# Autodesk Inventor assembly: Assembly1
(part 4 of 8)
- [Mate]: disk holder:94 ↔ Coil:188
- [Angle] (270 deg): disk holder:94 ↔ Coil:188
- [Mate]: disk holder:94 ↔ Coil:188
- [RevoluteJoint]: disk holder:95 ↔ coin:95
- [Angle] (-25 deg): disk holder:95 ↔ coin:95
- [Mate]: disk holder:95 ↔ Coil:189
- [Mate]: disk holder:95 ↔ Coil:189
- [Angle] (270 deg): disk holder:95 ↔ Coil:189
- [Mate]: disk holder:95 ↔ Coil:190
- [Angle] (270 deg): disk holder:95 ↔ Coil:190
- [Mate]: disk holder:95 ↔ Coil:190
- [RevoluteJoint]: disk holder:96 ↔ coin:96
- [Angle] (-25 deg): disk holder:96 ↔ coin:96
- [Mate]: disk holder:96 ↔ Coil:191
- [Mate]: disk holder:96 ↔ Coil:191
- [Angle] (270 deg): disk holder:96 ↔ Coil:191
- [Mate]: disk holder:96 ↔ Coil:192
- [Angle] (270 deg): disk holder:96 ↔ Coil:192
- [Mate]: disk holder:96 ↔ Coil:192
- [RevoluteJoint]: disk holder:97 ↔ coin:97
- [Angle] (-25 deg): disk holder:97 ↔ coin:97
- [Mate]: disk holder:97 ↔ Coil:193
- [Mate]: disk holder:97 ↔ Coil:193
- [Angle] (270 deg): disk holder:97 ↔ Coil:193
- [Mate]: disk holder:97 ↔ Coil:194
- [Angle] (270 deg): disk holder:97 ↔ Coil:194
- [Mate]: disk holder:97 ↔ Coil:194
- [RevoluteJoint]: disk holder:98 ↔ coin:98
- [Angle] (-25 deg): disk holder:98 ↔ coin:98
- [Mate]: disk holder:98 ↔ Coil:195
- [Mate]: disk holder:98 ↔ Coil:195
- [Angle] (270 deg): disk holder:98 ↔ Coil:195
- [Mate]: disk holder:98 ↔ Coil:196
- [Angle] (270 deg): disk holder:98 ↔ Coil:196
- [Mate]: disk holder:98 ↔ Coil:196
- [RevoluteJoint]: disk holder:99 ↔ coin:99
- [Angle] (-25 deg): disk holder:99 ↔ coin:99
- [Mate]: disk holder:99 ↔ Coil:197
- [Mate]: disk holder:99 ↔ Coil:197
- [Angle] (270 deg): disk holder:99 ↔ Coil:197
- [Mate]: disk holder:99 ↔ Coil:198
- [Angle] (270 deg): disk holder:99 ↔ Coil:198
- [Mate]: disk holder:99 ↔ Coil:198
- [RevoluteJoint]: disk holder:100 ↔ coin:100
- [Angle] (-25 deg): disk holder:100 ↔ coin:100
- [Mate]: disk holder:100 ↔ Coil:199
- [Mate]: disk holder:100 ↔ Coil:199
- [Angle] (270 deg): disk holder:100 ↔ Coil:199
- [Mate]: disk holder:100 ↔ Coil:200
- [Angle] (270 deg): disk holder:100 ↔ Coil:200
- [Mate]: disk holder:100 ↔ Coil:200
- [RevoluteJoint]: disk holder:101 ↔ coin:101
- [Angle] (-25 deg): disk holder:101 ↔ coin:101
- [Mate]: disk holder:101 ↔ Coil:201
- [Mate]: disk holder:101 ↔ Coil:201
- [Angle] (270 deg): disk holder:101 ↔ Coil:201
- [Mate]: disk holder:101 ↔ Coil:202
- [Angle] (270 deg): disk holder:101 ↔ Coil:202
- [Mate]: disk holder:101 ↔ Coil:202
- [RevoluteJoint]: disk holder:102 ↔ coin:102
- [Angle] (-25 deg): disk holder:102 ↔ coin:102
- [Mate]: disk holder:102 ↔ Coil:203
- [Mate]: disk holder:102 ↔ Coil:203
- [Angle] (270 deg): disk holder:102 ↔ Coil:203
- [Mate]: disk holder:102 ↔ Coil:204
- [Angle] (270 deg): disk holder:102 ↔ Coil:204
- [Mate]: disk holder:102 ↔ Coil:204
- Flush:135: FRAME:1 ↔ disk holder:94
- Mate:559: FRAME:1 ↔ disk holder:94
- Flush:136: disk holder:92 ↔ disk holder:94
- Flush:137: disk holder:92 ↔ disk holder:94
- Flush:138: disk holder:92 ↔ disk holder:93
- Flush:139: disk holder:92 ↔ disk holder:93
- Flush:140: disk holder:93 ↔ disk holder:95
- Flush:141: disk holder:93 ↔ disk holder:95
- Flush:142: disk holder:95 ↔ disk holder:96
- Flush:143: disk holder:95 ↔ disk holder:97
- Flush:144: disk holder:97 ↔ disk holder:98
- Flush:145: disk holder:98 ↔ disk holder:99
- Flush:146: disk holder:99 ↔ disk holder:100
- Flush:147: disk holder:95 ↔ disk holder:101
- Flush:148: disk holder:101 ↔ disk holder:102
- Flush:149: disk holder:93 ↔ disk holder:96
- Flush:150: disk holder:95 ↔ disk holder:97
- Flush:151: disk holder:95 ↔ disk holder:98
- Flush:152: disk holder:99 ↔ disk holder:100
- Flush:153: disk holder:100 ↔ disk holder:101
- Flush:154: disk holder:101 ↔ disk holder:102
- Flush:155: disk holder:98 ↔ disk holder:99
- Mate:560: FRAME:1 ↔ disk holder:94
- Mate:561: FRAME:1 ↔ disk holder:92
- Mate:562: FRAME:1 ↔ disk holder:93
- Mate:563: FRAME:1 ↔ disk holder:96
- Mate:564: FRAME:1 ↔ disk holder:97
- Mate:565: FRAME:1 ↔ disk holder:95
- Mate:566: FRAME:1 ↔ disk holder:98
- Mate:567: FRAME:1 ↔ disk holder:99
- Mate:568: FRAME:1 ↔ disk holder:100
- Mate:569: FRAME:1 ↔ disk holder:101
- Mate:570: FRAME:1 ↔ disk holder:102
- [RevoluteJoint]: disk holder:103 ↔ coin:103
- [Angle] (-25 deg): disk holder:103 ↔ coin:103
- [Mate]: disk holder:103 ↔ Coil:205
- [Mate]: disk holder:103 ↔ Coil:205
- [Angle] (270 deg): disk holder:103 ↔ Coil:205
- [Mate]: disk holder:103 ↔ Coil:206
- [Angle] (270 deg): disk holder:103 ↔ Coil:206
- [Mate]: disk holder:103 ↔ Coil:206
- [RevoluteJoint]: disk holder:104 ↔ coin:104
- [Angle] (-25 deg): disk holder:104 ↔ coin:104
- [Mate]: disk holder:104 ↔ Coil:207
- [Mate]: disk holder:104 ↔ Coil:207
- [Angle] (270 deg): disk holder:104 ↔ Coil:207
- [Mate]: disk holder:104 ↔ Coil:208
- [Angle] (270 deg): disk holder:104 ↔ Coil:208
- [Mate]: disk holder:104 ↔ Coil:208
- [RevoluteJoint]: disk holder:105 ↔ coin:105
- [Angle] (-25 deg): disk holder:105 ↔ coin:105
- [Mate]: disk holder:105 ↔ Coil:209
- [Mate]: disk holder:105 ↔ Coil:209
- [Angle] (270 deg): disk holder:105 ↔ Coil:209
- [Mate]: disk holder:105 ↔ Coil:210
- [Angle] (270 deg): disk holder:105 ↔ Coil:210
- [Mate]: disk holder:105 ↔ Coil:210
- [RevoluteJoint]: disk holder:106 ↔ coin:106
- [Angle] (-25 deg): disk holder:106 ↔ coin:106
- [Mate]: disk holder:106 ↔ Coil:211
- [Mate]: disk holder:106 ↔ Coil:211
- [Angle] (270 deg): disk holder:106 ↔ Coil:211
- [Mate]: disk holder:106 ↔ Coil:212
- [Angle] (270 deg): disk holder:106 ↔ Coil:212
- [Mate]: disk holder:106 ↔ Coil:212
- [RevoluteJoint]: disk holder:107 ↔ coin:107
- [Angle] (-25 deg): disk holder:107 ↔ coin:107
- [Mate]: disk holder:107 ↔ Coil:213
- [Mate]: disk holder:107 ↔ Coil:213
- [Angle] (270 deg): disk holder:107 ↔ Coil:213
- [Mate]: disk holder:107 ↔ Coil:214
- [Angle] (270 deg): disk holder:107 ↔ Coil:214
- [Mate]: disk holder:107 ↔ Coil:214
- [RevoluteJoint]: disk holder:108 ↔ coin:108
- [Angle] (-25 deg): disk holder:108 ↔ coin:108
- [Mate]: disk holder:108 ↔ Coil:215
- [Mate]: disk holder:108 ↔ Coil:215
- [Angle] (270 deg): disk holder:108 ↔ Coil:215
- [Mate]: disk holder:108 ↔ Coil:216
- [Angle] (270 deg): disk holder:108 ↔ Coil:216
- [Mate]: disk holder:108 ↔ Coil:216
- [RevoluteJoint]: disk holder:109 ↔ coin:109
- [Angle] (-25 deg): disk holder:109 ↔ coin:109
- [Mate]: disk holder:109 ↔ Coil:217
- [Mate]: disk holder:109 ↔ Coil:217
- [Angle] (270 deg): disk holder:109 ↔ Coil:217
- [Mate]: disk holder:109 ↔ Coil:218
- [Angle] (270 deg): disk holder:109 ↔ Coil:218
- [Mate]: disk holder:109 ↔ Coil:218
- [RevoluteJoint]: disk holder:110 ↔ coin:110
- [Angle] (-25 deg): disk holder:110 ↔ coin:110
- [Mate]: disk holder:110 ↔ Coil:219
- [Mate]: disk holder:110 ↔ Coil:219
- [Angle] (270 deg): disk holder:110 ↔ Coil:219
- [Mate]: disk holder:110 ↔ Coil:220
- [Angle] (270 deg): disk holder:110 ↔ Coil:220
- [Mate]: disk holder:110 ↔ Coil:220
- [RevoluteJoint]: disk holder:111 ↔ coin:111
- [Angle] (-25 deg): disk holder:111 ↔ coin:111
- [Mate]: disk holder:111 ↔ Coil:221
- [Mate]: disk holder:111 ↔ Coil:221
- [Angle] (270 deg): disk holder:111 ↔ Coil:221
- [Mate]: disk holder:111 ↔ Coil:222
- [Angle] (270 deg): disk holder:111 ↔ Coil:222
- [Mate]: disk holder:111 ↔ Coil:222
- Flush:156: FRAME:1 ↔ disk holder:107
- Mate:607: FRAME:1 ↔ disk holder:107
- Flush:157: disk holder:107 ↔ disk holder:108
- Flush:158: disk holder:108 ↔ disk holder:109
- Flush:159: disk holder:106 ↔ disk holder:108
- Flush:160: disk holder:106 ↔ disk holder:110
- Flush:161: disk holder:105 ↔ disk holder:110
- Flush:162: disk holder:105 ↔ disk holder:111
- Flush:163: disk holder:104 ↔ disk holder:111
- Flush:164: disk holder:103 ↔ disk holder:105
- Flush:165: disk holder:107 ↔ disk holder:108
- Flush:166: disk holder:106 ↔ disk holder:108
- Flush:167: disk holder:105 ↔ disk holder:106
- Flush:168: disk holder:106 ↔ disk holder:110
- Flush:169: disk holder:103 ↔ disk holder:107
- Flush:170: disk holder:107 ↔ disk holder:109
- Flush:171: disk holder:108 ↔ disk holder:111
- Flush:172: disk holder:104 ↔ disk holder:107
- Mate:608: FRAME:1 ↔ disk holder:109
- Mate:609: FRAME:1 ↔ disk holder:104
- Mate:610: FRAME:1 ↔ disk holder:111
- Mate:611: FRAME:1 ↔ disk holder:103
- Mate:612: FRAME:1 ↔ disk holder:105
- Mate:613: FRAME:1 ↔ disk holder:107
- Mate:614: FRAME:1 ↔ disk holder:110
- Mate:615: FRAME:1 ↔ disk holder:106
- Mate:616: FRAME:1 ↔ disk holder:108
- [RevoluteJoint]: disk holder:112 ↔ coin:112
- [Angle] (-25 deg): disk holder:112 ↔ coin:112
- [Mate]: disk holder:112 ↔ Coil:223
- [Mate]: disk holder:112 ↔ Coil:223
- [Angle] (270 deg): disk holder:112 ↔ Coil:223
- [Mate]: disk holder:112 ↔ Coil:224
- [Angle] (270 deg): disk holder:112 ↔ Coil:224
- [Mate]: disk holder:112 ↔ Coil:224
- [RevoluteJoint]: disk holder:113 ↔ coin:113
- [Angle] (-25 deg): disk holder:113 ↔ coin:113
- [Mate]: disk holder:113 ↔ Coil:225
- [Mate]: disk holder:113 ↔ Coil:225
- [Angle] (270 deg): disk holder:113 ↔ Coil:225
- [Mate]: disk holder:113 ↔ Coil:226
- [Angle] (270 deg): disk holder:113 ↔ Coil:226
- [Mate]: disk holder:113 ↔ Coil:226
- [RevoluteJoint]: disk holder:114 ↔ coin:114
- [Angle] (-25 deg): disk holder:114 ↔ coin:114
- [Mate]: disk holder:114 ↔ Coil:227
- [Mate]: disk holder:114 ↔ Coil:227
- [Angle] (270 deg): disk holder:114 ↔ Coil:227
- [Mate]: disk holder:114 ↔ Coil:228
- [Angle] (270 deg): disk holder:114 ↔ Coil:228
- [Mate]: disk holder:114 ↔ Coil:228
- [RevoluteJoint]: disk holder:115 ↔ coin:115
- [Angle] (-25 deg): disk holder:115 ↔ coin:115
- [Mate]: disk holder:115 ↔ Coil:229
- [Mate]: disk holder:115 ↔ Coil:229
- [Angle] (270 deg): disk holder:115 ↔ Coil:229
- [Mate]: disk holder:115 ↔ Coil:230
- [Angle] (270 deg): disk holder:115 ↔ Coil:230
- [Mate]: disk holder:115 ↔ Coil:230
- [RevoluteJoint]: disk holder:116 ↔ coin:116
- [Angle] (-25 deg): disk holder:116 ↔ coin:116
- [Mate]: disk holder:116 ↔ Coil:231
- [Mate]: disk holder:116 ↔ Coil:231
- [Angle] (270 deg): disk holder:116 ↔ Coil:231
- [Mate]: disk holder:116 ↔ Coil:232
- [Angle] (270 deg): disk holder:116 ↔ Coil:232
- [Mate]: disk holder:116 ↔ Coil:232
- [RevoluteJoint]: disk holder:117 ↔ coin:117
- [Angle] (-25 deg): disk holder:117 ↔ coin:117
- [Mate]: disk holder:117 ↔ Coil:233
- [Mate]: disk holder:117 ↔ Coil:233
- [Angle] (270 deg): disk holder:117 ↔ Coil:233
- [Mate]: disk holder:117 ↔ Coil:234
- [Angle] (270 deg): disk holder:117 ↔ Coil:234
- [Mate]: disk holder:117 ↔ Coil:234
- [RevoluteJoint]: disk holder:118 ↔ coin:118
- [Angle] (-25 deg): disk holder:118 ↔ coin:118
- [Mate]: disk holder:118 ↔ Coil:235
- [Mate]: disk holder:118 ↔ Coil:235
- [Angle] (270 deg): disk holder:118 ↔ Coil:235
- [Mate]: disk holder:118 ↔ Coil:236
- [Angle] (270 deg): disk holder:118 ↔ Coil:236
- [Mate]: disk holder:118 ↔ Coil:236
- [RevoluteJoint]: disk holder:119 ↔ coin:119
- [Angle] (-25 deg): disk holder:119 ↔ coin:119
- [Mate]: disk holder:119 ↔ Coil:237
- [Mate]: disk holder:119 ↔ Coil:237
- [Angle] (270 deg): disk holder:119 ↔ Coil:237
- [Mate]: disk holder:119 ↔ Coil:238
- [Angle] (270 deg): disk holder:119 ↔ Coil:238
- [Mate]: disk holder:119 ↔ Coil:238
- [RevoluteJoint]: disk holder:120 ↔ coin:120
- [Angle] (-25 deg): disk holder:120 ↔ coin:120
- [Mate]: disk holder:120 ↔ Coil:239
- [Mate]: disk holder:120 ↔ Coil:239
- [Angle] (270 deg): disk holder:120 ↔ Coil:239
- [Mate]: disk holder:120 ↔ Coil:240
- [Angle] (270 deg): disk holder:120 ↔ Coil:240
- [Mate]: disk holder:120 ↔ Coil:240
- [RevoluteJoint]: disk holder:121 ↔ coin:121
- [Angle] (-25 deg): disk holder:121 ↔ coin:121
- [Mate]: disk holder:121 ↔ Coil:241
- [Mate]: disk holder:121 ↔ Coil:241
- [Angle] (270 deg): disk holder:121 ↔ Coil:241
- [Mate]: disk holder:121 ↔ Coil:242
- [Angle] (270 deg): disk holder:121 ↔ Coil:242
- [Mate]: disk holder:121 ↔ Coil:242
- Flush:173: FRAME:1 ↔ disk holder:112
- Mate:657: FRAME:1 ↔ disk holder:112
- Flush:174: disk holder:112 ↔ disk holder:113
- Flush:175: disk holder:113 ↔ disk holder:114
- Flush:176: disk holder:114 ↔ disk holder:119
- Flush:177: disk holder:115 ↔ disk holder:119
- Flush:178: disk holder:115 ↔ disk holder:116
- Flush:179: disk holder:116 ↔ disk holder:120
- Flush:180: disk holder:120 ↔ disk holder:121
- Flush:181: disk holder:117 ↔ disk holder:121
- Flush:182: disk holder:112 ↔ disk holder:113
- Flush:183: disk holder:113 ↔ disk holder:114
- Flush:184: disk holder:114 ↔ disk holder:119
- Flush:185: disk holder:115 ↔ disk holder:119
- Flush:186: disk holder:115 ↔ disk holder:116
- Flush:187: disk holder:116 ↔ disk holder:120
- Flush:188: disk holder:116 ↔ disk holder:121
- Flush:189: disk holder:117 ↔ disk holder:121
- Flush:190: disk holder:117 ↔ disk holder:118
- Mate:658: FRAME:1 ↔ disk holder:112
- Mate:659: FRAME:1 ↔ disk holder:113
- Mate:660: FRAME:1 ↔ disk holder:114
- Mate:661: FRAME:1 ↔ disk holder:119
- Mate:662: FRAME:1 ↔ disk holder:115
- Mate:663: FRAME:1 ↔ disk holder:120
- Mate:664: FRAME:1 ↔ disk holder:116
- Mate:665: FRAME:1 ↔ disk holder:121
- Mate:666: FRAME:1 ↔ disk holder:117
- Mate:667: FRAME:1 ↔ disk holder:118
- Flush:191: disk holder:117 ↔ disk holder:118
- [RevoluteJoint]: disk holder:122 ↔ coin:122
- [Angle] (-25 deg): disk holder:122 ↔ coin:122
- [Mate]: disk holder:122 ↔ Coil:243
- [Mate]: disk holder:122 ↔ Coil:243
- [Angle] (270 deg): disk holder:122 ↔ Coil:243
- [Mate]: disk holder:122 ↔ Coil:244
- [Angle] (270 deg): disk holder:122 ↔ Coil:244
- [Mate]: disk holder:122 ↔ Coil:244
- [RevoluteJoint]: disk holder:123 ↔ coin:123
- [Angle] (-25 deg): disk holder:123 ↔ coin:123
- [Mate]: disk holder:123 ↔ Coil:245
- [Mate]: disk holder:123 ↔ Coil:245
- [Angle] (270 deg): disk holder:123 ↔ Coil:245
- [Mate]: disk holder:123 ↔ Coil:246
- [Angle] (270 deg): disk holder:123 ↔ Coil:246
- [Mate]: disk holder:123 ↔ Coil:246
- [RevoluteJoint]: disk holder:124 ↔ coin:124
- [Angle] (-25 deg): disk holder:124 ↔ coin:124
- [Mate]: disk holder:124 ↔ Coil:247
- [Mate]: disk holder:124 ↔ Coil:247
- [Angle] (270 deg): disk holder:124 ↔ Coil:247
- [Mate]: disk holder:124 ↔ Coil:248
- [Angle] (270 deg): disk holder:124 ↔ Coil:248
- [Mate]: disk holder:124 ↔ Coil:248
- [RevoluteJoint]: disk holder:125 ↔ coin:125
- [Angle] (-25 deg): disk holder:125 ↔ coin:125
- [Mate]: disk holder:125 ↔ Coil:249
- [Mate]: disk holder:125 ↔ Coil:249
- [Angle] (270 deg): disk holder:125 ↔ Coil:249
- [Mate]: disk holder:125 ↔ Coil:250
- [Angle] (270 deg): disk holder:125 ↔ Coil:250
- [Mate]: disk holder:125 ↔ Coil:250
- [RevoluteJoint]: disk holder:126 ↔ coin:126
- [Angle] (-25 deg): disk holder:126 ↔ coin:126
- [Mate]: disk holder:126 ↔ Coil:251
- [Mate]: disk holder:126 ↔ Coil:251
- [Angle] (270 deg): disk holder:126 ↔ Coil:251
- [Mate]: disk holder:126 ↔ Coil:252
- [Angle] (270 deg): disk holder:126 ↔ Coil:252
- [Mate]: disk holder:126 ↔ Coil:252
- [RevoluteJoint]: disk holder:127 ↔ coin:127
- [Angle] (-25 deg): disk holder:127 ↔ coin:127
- [Mate]: disk holder:127 ↔ Coil:253
- [Mate]: disk holder:127 ↔ Coil:253
- [Angle] (270 deg): disk holder:127 ↔ Coil:253
- [Mate]: disk holder:127 ↔ Coil:254
- [Angle] (270 deg): disk holder:127 ↔ Coil:254
- [Mate]: disk holder:127 ↔ Coil:254
- [RevoluteJoint]: disk holder:128 ↔ coin:128
- [Angle] (-25 deg): disk holder:128 ↔ coin:128
- [Mate]: disk holder:128 ↔ Coil:255
- [Mate]: disk holder:128 ↔ Coil:255
- [Angle] (270 deg): disk holder:128 ↔ Coil:255
- [Mate]: disk holder:128 ↔ Coil:256
- [Angle] (270 deg): disk holder:128 ↔ Coil:256
- [Mate]: disk holder:128 ↔ Coil:256
- Mate:696: disk holder:127 ↔ disk holder:128
- Mate:697: disk holder:126 ↔ disk holder:127
- Mate:698: disk holder:125 ↔ disk holder:126
- Mate:699: disk holder:124 ↔ disk holder:125
- Mate:700: disk holder:123 ↔ disk holder:124
- Mate:701: disk holder:122 ↔ disk holder:123
- Flush:192: FRAME:1 ↔ disk holder:122
- Flush:193: disk holder:122 ↔ disk holder:123
- Flush:194: disk holder:123 ↔ disk holder:124
- Flush:195: disk holder:123 ↔ disk holder:125
- Flush:196: disk holder:125 ↔ disk holder:126
- Flush:197: disk holder:126 ↔ disk holder:127
- Flush:198: disk holder:127 ↔ disk holder:128
- Mate:702: FRAME:1 ↔ disk holder:122
- Mate:703: FRAME:1 ↔ disk holder:122
- Mate:704: FRAME:1 ↔ disk holder:123
- Mate:705: FRAME:1 ↔ disk holder:124
- Mate:706: FRAME:1 ↔ disk holder:125
- Mate:707: FRAME:1 ↔ disk holder:126
- Mate:708: FRAME:1 ↔ disk holder:127
- Mate:709: FRAME:1 ↔ disk holder:128
- [RevoluteJoint]: disk holder:129 ↔ coin:129
- [Angle] (-25 deg): disk holder:129 ↔ coin:129
- [Mate]: disk holder:129 ↔ Coil:257
- [Mate]: disk holder:129 ↔ Coil:257
- [Angle] (270 deg): disk holder:129 ↔ Coil:257
- [Mate]: disk holder:129 ↔ Coil:258
- [Angle] (270 deg): disk holder:129 ↔ Coil:258
- [Mate]: disk holder:129 ↔ Coil:258
- [RevoluteJoint]: disk holder:130 ↔ coin:130
- [Angle] (-25 deg): disk holder:130 ↔ coin:130
- [Mate]: disk holder:130 ↔ Coil:259
- [Mate]: disk holder:130 ↔ Coil:259
- [Angle] (270 deg): disk holder:130 ↔ Coil:259
- [Mate]: disk holder:130 ↔ Coil:260
- [Angle] (270 deg): disk holder:130 ↔ Coil:260
- [Mate]: disk holder:130 ↔ Coil:260
- [RevoluteJoint]: disk holder:131 ↔ coin:131
- [Angle] (-25 deg): disk holder:131 ↔ coin:131
- [Mate]: disk holder:131 ↔ Coil:261
- [Mate]: disk holder:131 ↔ Coil:261
- [Angle] (270 deg): disk holder:131 ↔ Coil:261
- [Mate]: disk holder:131 ↔ Coil:262
- [Angle] (270 deg): disk holder:131 ↔ Coil:262
- [Mate]: disk holder:131 ↔ Coil:262
- [RevoluteJoint]: disk holder:132 ↔ coin:132
- [Angle] (-25 deg): disk holder:132 ↔ coin:132
- [Mate]: disk holder:132 ↔ Coil:263
- [Mate]: disk holder:132 ↔ Coil:263
- [Angle] (270 deg): disk holder:132 ↔ Coil:263
- [Mate]: disk holder:132 ↔ Coil:264
- [Angle] (270 deg): disk holder:132 ↔ Coil:264
- [Mate]: disk holder:132 ↔ Coil:264
- [RevoluteJoint]: disk holder:133 ↔ coin:133
- [Angle] (-25 deg): disk holder:133 ↔ coin:133
- [Mate]: disk holder:133 ↔ Coil:265
- [Mate]: disk holder:133 ↔ Coil:265
- [Angle] (270 deg): disk holder:133 ↔ Coil:265
- [Mate]: disk holder:133 ↔ Coil:266
- [Angle] (270 deg): disk holder:133 ↔ Coil:266
- [Mate]: disk holder:133 ↔ Coil:266
- [RevoluteJoint]: disk holder:134 ↔ coin:134
- [Angle] (-25 deg): disk holder:134 ↔ coin:134
- [Mate]: disk holder:134 ↔ Coil:267
- [Mate]: disk holder:134 ↔ Coil:267
- [Angle] (270 deg): disk holder:134 ↔ Coil:267
- [Mate]: disk holder:134 ↔ Coil:268
- [Angle] (270 deg): disk holder:134 ↔ Coil:268
- [Mate]: disk holder:134 ↔ Coil:268
- [RevoluteJoint]: disk holder:135 ↔ coin:135
- [Angle] (-25 deg): disk holder:135 ↔ coin:135
- [Mate]: disk holder:135 ↔ Coil:269
- [Mate]: disk holder:135 ↔ Coil:269
- [Angle] (270 deg): disk holder:135 ↔ Coil:269
- [Mate]: disk holder:135 ↔ Coil:270
- [Angle] (270 deg): disk holder:135 ↔ Coil:270
- [Mate]: disk holder:135 ↔ Coil:270
- [RevoluteJoint]: disk holder:136 ↔ coin:136
- [Angle] (-25 deg): disk holder:136 ↔ coin:136
- [Mate]: disk holder:136 ↔ Coil:271
- [Mate]: disk holder:136 ↔ Coil:271
- [Angle] (270 deg): disk holder:136 ↔ Coil:271
- [Mate]: disk holder:136 ↔ Coil:272
- [Angle] (270 deg): disk holder:136 ↔ Coil:272
- [Mate]: disk holder:136 ↔ Coil:272
- Flush:199: disk holder:129 ↔ disk holder:130
- Flush:200: disk holder:130 ↔ disk holder:131
- Flush:201: disk holder:131 ↔ disk holder:132
- Flush:202: disk holder:132 ↔ disk holder:133
- Flush:203: disk holder:133 ↔ disk holder:134
- Flush:204: disk holder:134 ↔ disk holder:135
- Flush:205: disk holder:135 ↔ disk holder:136
- Flush:206: disk holder:135 ↔ disk holder:136
- Flush:207: disk holder:134 ↔ disk holder:135
- Flush:208: disk holder:133 ↔ disk holder:134
- Flush:209: disk holder:132 ↔ disk holder:133
- Flush:210: disk holder:131 ↔ disk holder:132
- Flush:211: disk holder:130 ↔ disk holder:131
- Flush:212: disk holder:129 ↔ disk holder:130
- Mate:742: FRAME:1 ↔ disk holder:129
- Mate:743: FRAME:1 ↔ disk holder:129
- Mate:744: FRAME:1 ↔ disk holder:130
- Mate:745: FRAME:1 ↔ disk holder:131
- Mate:746: FRAME:1 ↔ disk holder:132